# Autodesk Inventor assembly: Camera Side Panel Assembly
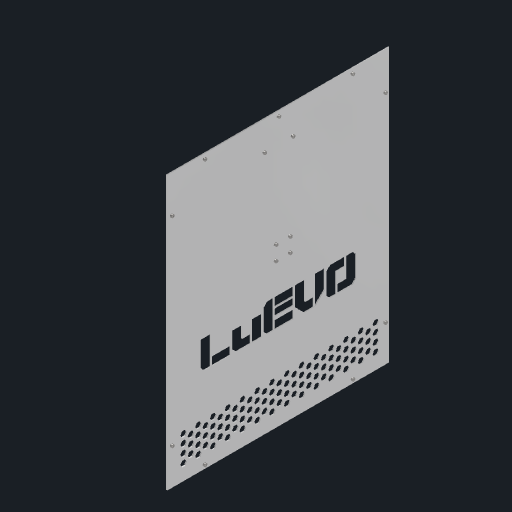
[picture p0: Inventor's stored thumbnail of the model, 512x512]
Saved by Autodesk Inventor 2023.1 (Build 271208000, 208)
## iProperties
Created: 2023-02-06
Part Number: Camera Side Panel Assembly
Document SubType Name: Assembly
Designer: remop
Author: remop
## Documents named in this file (8)
- C:\Users\remop\OneDrive\Documents\Inventor\3D Printers\LuEVO\Mk5_FullKinematic\Frame and Panels\Camera Side Panel Assembly.iam
- C:\Users\remop\OneDrive\Documents\Inventor\3D Printers\LuEVO\Mk5_FullKinematic\Frame and Panels\Camera Side Panel.ipt
- C:\Users\remop\OneDrive\Documents\Inventor\Content Center Files\R2023\en-US\AS 1420\AS 1420 - 1973 - M3 x 6.ipt
- C:\Users\remop\OneDrive\Documents\Inventor\3D Printers\LuEVO\Mk5_FullKinematic\Filament Spool Holder.ipt
- C:\Users\remop\OneDrive\Documents\Inventor\Content Center Files\R2023\en-US\AS 1420\AS 1420 - 1973 - M3 x 12.ipt
- C:\Users\remop\OneDrive\Documents\Inventor\3D Printers\LuEVO\Mk5_FullKinematic\Electronics\Waveshare Cam Holder - Overview.ipt
- C:\Users\remop\OneDrive\Documents\Inventor\3D Printers\LuEVO\Mk5_FullKinematic\Electronics\Waveshare OV5640.ipt
- C:\Users\remop\OneDrive\Documents\Inventor\Content Center Files\R2023\en-US\AS 1420\AS 1420 - 1973 - M3 x 8.ipt
## Components (19 placed, 7 different names)
1. Camera Side Panel:1 — Insert:1, Insert:2, Insert:3, Insert:4, Insert:5, Insert:6, Insert:7, Insert:8, Insert:9, Rigid:1, Insert:10, Insert:11, Insert:12, Insert:13, Rigid:3, Insert:14, Insert:15
2. AS 1420 - Metric M3 x 6:1 — Insert:1
3. AS 1420 - Metric M3 x 6:2 — Insert:2
4. AS 1420 - Metric M3 x 6:3 — Insert:3
5. AS 1420 - Metric M3 x 6:4 — Insert:4
6. AS 1420 - Metric M3 x 6:5 — Insert:5
7. AS 1420 - Metric M3 x 6:6 — Insert:6
8. AS 1420 - Metric M3 x 6:7 — Insert:7
9. AS 1420 - Metric M3 x 6:8 — Insert:8
10. AS 1420 - Metric M3 x 6:9 — Insert:9
11. Filament Spool Holder:1 — Rigid:1
12. AS 1420 - Metric M3 x 12:1 — Insert:10
13. AS 1420 - Metric M3 x 12:2 — Insert:11
14. AS 1420 - Metric M3 x 12:3 — Insert:12
15. AS 1420 - Metric M3 x 12:4 — Insert:13
16. Waveshare Cam Holder - Overview:1 — Rigid:2, Rigid:3
17. Waveshare OV5640:1 — Rigid:2
18. AS 1420 - Metric M3 x 8:1 — Insert:14
19. AS 1420 - Metric M3 x 8:2 — Insert:15
## Relationships (18: Insert 15, WeldJoint 3)
- Insert:1: Camera Side Panel:1 ↔ AS 1420 - Metric M3 x 6:1
- Insert:2: Camera Side Panel:1 ↔ AS 1420 - Metric M3 x 6:2
- Insert:3: Camera Side Panel:1 ↔ AS 1420 - Metric M3 x 6:3
- Insert:4: Camera Side Panel:1 ↔ AS 1420 - Metric M3 x 6:4
- Insert:5: Camera Side Panel:1 ↔ AS 1420 - Metric M3 x 6:5
- Insert:6: Camera Side Panel:1 ↔ AS 1420 - Metric M3 x 6:6
- Insert:7: Camera Side Panel:1 ↔ AS 1420 - Metric M3 x 6:7
- Insert:8: Camera Side Panel:1 ↔ AS 1420 - Metric M3 x 6:8
- Insert:9: Camera Side Panel:1 ↔ AS 1420 - Metric M3 x 6:9
- Rigid:1 [WeldJoint]: Camera Side Panel:1 ↔ Filament Spool Holder:1
- Insert:10: Camera Side Panel:1 ↔ AS 1420 - Metric M3 x 12:1
- Insert:11: Camera Side Panel:1 ↔ AS 1420 - Metric M3 x 12:2
- Insert:12: Camera Side Panel:1 ↔ AS 1420 - Metric M3 x 12:3
- Insert:13: Camera Side Panel:1 ↔ AS 1420 - Metric M3 x 12:4
- Rigid:2 [WeldJoint]: Waveshare Cam Holder - Overview:1 ↔ Waveshare OV5640:1
- Rigid:3 [WeldJoint]: Camera Side Panel:1 ↔ Waveshare Cam Holder - Overview:1
- Insert:14: Camera Side Panel:1 ↔ AS 1420 - Metric M3 x 8:1
- Insert:15: Camera Side Panel:1 ↔ AS 1420 - Metric M3 x 8:2
